# Autodesk Inventor assembly: MX-64AT_AR_contreaxe
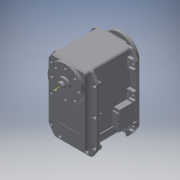
[picture p0: Inventor's stored thumbnail of the model, 180x180]
Saved by Autodesk Inventor 2018 (Build 220112000, 112)
## iProperties
Created: 2017-01-31
Part Number: MX-64AT_AR_contreaxe
Document SubType Name: Assembly
Designer: steve
Mass: 140.592 g
Surface Area: 175.398 cm^2
Volume: 73.6513 cm^3
Density: 1.90889 g/cm^3
Author: steve
## Documents named in this file (5)
- C:\Users\User\Downloads\robot\MX-64AT_AR_contreaxe.iam
- C:\Users\User\Downloads\robot\MX-64AT_AR.ipt
- C:\Users\User\Downloads\robot\RX64-CAP.ipt
- C:\Users\User\Downloads\robot\HN05-i101.ipt
- C:\Users\User\Downloads\robot\MF128ZZ.ipt
## Components (4 placed, 4 different names)
1. MX-64AT_AR:1 — Flush:1
2. RX64-CAP:1
3. HN05-i101:1 — Flush:1
4. MF128ZZ:1
## Relationships (6: Mate 5, Flush 1)
- [Mate]: MX-64AT_AR:1 ↔ HN05-i101:1
- [Mate]: HN05-i101:1 ↔ MF128ZZ:1
- [Mate]: RX64-CAP:1 ↔ MF128ZZ:1
- [Mate]: RX64-CAP:1 ↔ MF128ZZ:1
- [Mate]: MX-64AT_AR:1 ↔ MF128ZZ:1
- Flush:1 (-3 mm): MX-64AT_AR:1 ↔ HN05-i101:1
